# Autodesk Inventor assembly: worm gear
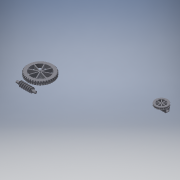
[picture p0: Inventor's stored thumbnail of the model, 180x180]
Saved by Autodesk Inventor 2016 (Build 200138000, 138)
## iProperties
Created: 2016-07-27
Part Number: worm gear
Document SubType Name: Assembly
Designer: Admin
Author: Admin
## Documents named in this file (5)
- C:\Users\Admin\Documents\diseños autodesk dimer\worm gear.iam
- C:\Users\Admin\Documents\diseños autodesk dimer\worm gear\Design Accelerator\Worm Gears2.iam
- C:\Users\Admin\Documents\diseños autodesk dimer\worm gear\Design Accelerator\Worm Gears3.iam
- C:\Users\Admin\Documents\diseños autodesk dimer\worm gear\Design Accelerator\Spur Gears1.iam
- C:\Users\Admin\Documents\diseños autodesk dimer\worm gear\Design Accelerator\Spur Gears2.iam
## Components (4 placed, 2 different names)
1. Worm Gears:1 [sub-assembly]
2. Worm Gears:2 [sub-assembly] — Mate:1, Flush:1, Mate:2
3. Spur Gears:1 [sub-assembly] — Mate:1, Flush:1, Mate:2, Flush:2
4. Spur Gears:2 [sub-assembly] — Flush:2
## Relationships (4: Mate 2, Flush 2)
- Mate:1: Worm Gears:2 ↔ Spur Gears:1
- Flush:1: Worm Gears:2 ↔ Spur Gears:1
- Mate:2: Worm Gears:2 ↔ Spur Gears:1
- Flush:2: Spur Gears:1 ↔ Spur Gears:2
